# Autodesk Inventor assembly: Base
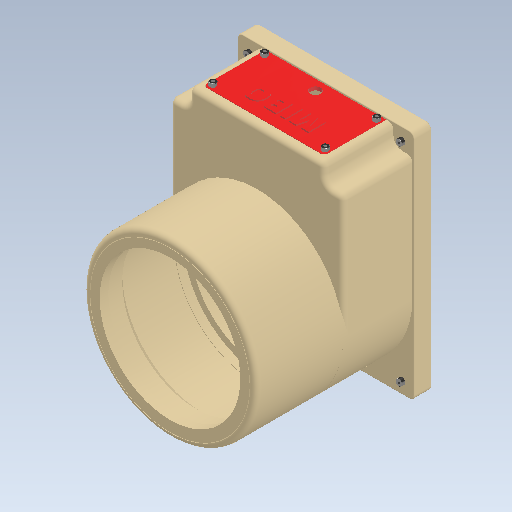
[picture p0: Inventor's stored thumbnail of the model, 512x512]
Saved by Autodesk Inventor 2021 (Build 250183000, 183)
## iProperties
Created: 2020-02-11
Part Number: Base
Document SubType Name: Assembly
Designer: JochenAlt
Author: JochenAlt
## Documents named in this file (6)
- C:\Users\Jochen Alt\Documents\Daten\Projects\MiniBot\CAD\Base.iam
- C:\Users\Jochen Alt\Documents\Daten\Projects\MiniBot\CAD\Base.ipt
- C:\Users\Jochen Alt\Documents\Daten\Projects\MiniBot\CAD\extern\electronics\Odroid C2\ODroid C2.iam
- D:\Projects\MiniBot\CAD\extern\DIN 912\DIN 912 - M2 x 0.4 x 10 x 9.ipt
- D:\Projects\MiniBot\CAD\extern\DIN 912\DIN 912 - M2 x 0,4 x 20 x 19.ipt
- D:\Projects\MiniBot\CAD\extern\DIN 912\DIN 912 - M2 x 0,4 x 6 x 5.ipt
## Components (23 placed, 5 different names)
1. Base:1 — Passend:1, Winkel:1, Insert:5, Insert:6, Insert:7, Insert:8, Insert:9, Insert:10, Insert:11, Insert:12, Insert:13, Insert:18, Insert:19, Insert:20, Insert:21
2. ODroid C2:1 [sub-assembly] — Passend:1, Winkel:1
3. DIN 912 - replaced by DIN EN ISO 4762 M2 x 10:1
4. DIN 912 - replaced by DIN EN ISO 4762 M2 x 10:2
5. DIN 912 - replaced by DIN EN ISO 4762 M2 x 10:3
6. DIN 912 - replaced by DIN EN ISO 4762 M2 x 10:4
7. DIN 912 - replaced by DIN EN ISO 4762 M2 x 20:1 — Insert:5
8. DIN 912 - replaced by DIN EN ISO 4762 M2 x 20:2 — Insert:6
9. DIN 912 - replaced by DIN EN ISO 4762 M2 x 20:3 — Insert:7
10. DIN 912 - replaced by DIN EN ISO 4762 M2 x 20:4 — Insert:8
11. DIN 912 - replaced by DIN EN ISO 4762 M2 x 20:5 — Insert:9
12. DIN 912 - replaced by DIN EN ISO 4762 M2 x 20:6 — Insert:10
13. DIN 912 - replaced by DIN EN ISO 4762 M2 x 20:7 — Insert:11
14. DIN 912 - replaced by DIN EN ISO 4762 M2 x 20:8 — Insert:12
15. DIN 912 - replaced by DIN EN ISO 4762 M2 x 20:9 — Insert:13
16. DIN 912 - replaced by DIN EN ISO 4762 M2 x 10:5
17. DIN 912 - replaced by DIN EN ISO 4762 M2 x 10:6
18. DIN 912 - replaced by DIN EN ISO 4762 M2 x 10:7
19. DIN 912 - replaced by DIN EN ISO 4762 M2 x 10:8
20. DIN 912 - replaced by DIN EN ISO 4762 M2 x 6:1 — Insert:18
21. DIN 912 - replaced by DIN EN ISO 4762 M2 x 6:2 — Insert:19
22. DIN 912 - replaced by DIN EN ISO 4762 M2 x 6:3 — Insert:20
23. DIN 912 - replaced by DIN EN ISO 4762 M2 x 6:4 — Insert:21
## Relationships (23: Insert 21, Mate 1, Angle 1)
- Passend:1 [Mate] (5 mm): Base:1 ↔ ODroid C2:1
- Winkel:1 [Angle] (0 deg): Base:1 ↔ ODroid C2:1
- [Insert]: Base:1 ↔ DIN 912 - replaced by DIN EN ISO 4762 M2 x 10:1
- [Insert]: Base:1 ↔ DIN 912 - replaced by DIN EN ISO 4762 M2 x 10:2
- [Insert]: Base:1 ↔ DIN 912 - replaced by DIN EN ISO 4762 M2 x 10:3
- [Insert]: Base:1 ↔ DIN 912 - replaced by DIN EN ISO 4762 M2 x 10:4
- Insert:5: Base:1 ↔ DIN 912 - replaced by DIN EN ISO 4762 M2 x 20:1
- Insert:6: Base:1 ↔ DIN 912 - replaced by DIN EN ISO 4762 M2 x 20:2
- Insert:7: Base:1 ↔ DIN 912 - replaced by DIN EN ISO 4762 M2 x 20:3
- Insert:8: Base:1 ↔ DIN 912 - replaced by DIN EN ISO 4762 M2 x 20:4
- Insert:9: Base:1 ↔ DIN 912 - replaced by DIN EN ISO 4762 M2 x 20:5
- Insert:10: Base:1 ↔ DIN 912 - replaced by DIN EN ISO 4762 M2 x 20:6
- Insert:11: Base:1 ↔ DIN 912 - replaced by DIN EN ISO 4762 M2 x 20:7
- Insert:12: Base:1 ↔ DIN 912 - replaced by DIN EN ISO 4762 M2 x 20:8
- Insert:13: Base:1 ↔ DIN 912 - replaced by DIN EN ISO 4762 M2 x 20:9
- [Insert]: Base:1 ↔ DIN 912 - replaced by DIN EN ISO 4762 M2 x 10:5
- [Insert]: Base:1 ↔ DIN 912 - replaced by DIN EN ISO 4762 M2 x 10:6
- [Insert]: Base:1 ↔ DIN 912 - replaced by DIN EN ISO 4762 M2 x 10:7
- [Insert]: Base:1 ↔ DIN 912 - replaced by DIN EN ISO 4762 M2 x 10:8
- Insert:18: Base:1 ↔ DIN 912 - replaced by DIN EN ISO 4762 M2 x 6:1
- Insert:19: Base:1 ↔ DIN 912 - replaced by DIN EN ISO 4762 M2 x 6:2
- Insert:20: Base:1 ↔ DIN 912 - replaced by DIN EN ISO 4762 M2 x 6:3
- Insert:21: Base:1 ↔ DIN 912 - replaced by DIN EN ISO 4762 M2 x 6:4
